# Autodesk Inventor assembly: Assembly_ThiHK
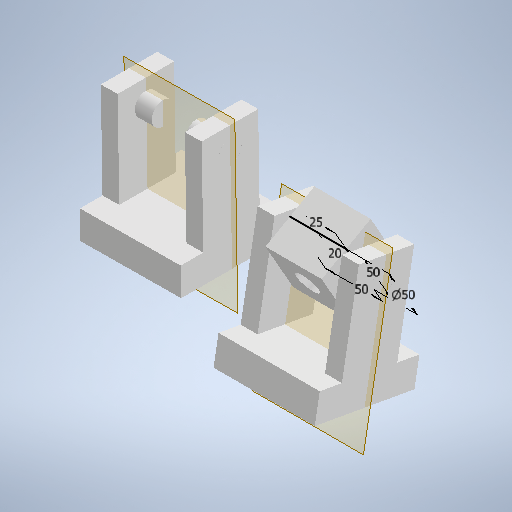
[picture p0: Inventor's stored thumbnail of the model, 512x512]
Saved by Autodesk Inventor 2025.2 (Build 292293000, 293)
## iProperties
Created: 2024-12-05
Part Number: Assembly_ThiHK
Document SubType Name: Assembly
Designer: hongquan
Author: hongquan
## Documents named in this file (4)
- C:\Users\hongquan\Documents\GitHub\Optimal-Design-Robot\Inventor\Hopgiamtoc\Assembly_ThiHK.iam
- C:\Users\hongquan\Documents\GitHub\Optimal-Design-Robot\Inventor\Hopgiamtoc\CT_01.ipt
- C:\Users\hongquan\Documents\GitHub\Optimal-Design-Robot\Inventor\Hopgiamtoc\CT_02.ipt
- C:\Users\hongquan\Documents\GitHub\Optimal-Design-Robot\Inventor\Hopgiamtoc\CT_03.ipt
## Components (7 placed, 3 different names)
1. CT_01:1 — Mate:3, Mate:4, Flush:1, Mate:6, Mate:10, Flush:4
2. CT_01:2 — Mate:1, Mate:2, Mate:7, Mate:8, Flush:2, Flush:3
3. CT_02:1 — Mate:5, Mate:6, Mate:9, Mate:11
4. CT_03:1 — Mate:1, Mate:7, Mate:8, Flush:3, Mate:11
5. CT_03:2 — Mate:3, Flush:4
6. CT_03:3 — Mate:4, Mate:5, Flush:1, Mate:10
7. CT_03:4 — Mate:2, Flush:2, Mate:9
## Relationships (15: Mate 11, Flush 4)
- Mate:1: CT_01:2 ↔ CT_03:1
- Mate:2: CT_01:2 ↔ CT_03:4
- Mate:3: CT_01:1 ↔ CT_03:2
- Mate:4: CT_01:1 ↔ CT_03:3
- Mate:5: CT_02:1 ↔ CT_03:3
- Flush:1: CT_01:1 ↔ CT_03:3
- Mate:6 (5 mm): CT_01:1 ↔ CT_02:1
- Mate:7: CT_01:2 ↔ CT_03:1
- Mate:8: CT_01:2 ↔ CT_03:1
- Flush:2: CT_01:2 ↔ CT_03:4
- Flush:3: CT_01:2 ↔ CT_03:1
- Mate:9: CT_02:1 ↔ CT_03:4
- Mate:10: CT_01:1 ↔ CT_03:3
- Flush:4: CT_01:1 ↔ CT_03:2
- Mate:11: CT_02:1 ↔ CT_03:1
